# Autodesk Inventor assembly: Сборка
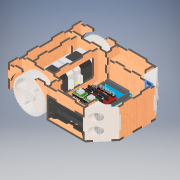
[picture p0: Inventor's stored thumbnail of the model, 180x180]
Saved by Autodesk Inventor 2019 (Build 230136000, 136)
## iProperties
Created: 2020-12-06
Part Number: Сборка
Material: Типовые
Document SubType Name: Assembly
Designer: Professional
Author: Professional
## Documents named in this file (25)
- C:\Users\Professional\Desktop\DeliveryBot\3dModels\assembly.iam
- C:\Users\Professional\Desktop\DeliveryBot\3dModels\Components\42BYGH47.ipt
- C:\Users\Professional\Desktop\DeliveryBot\3dModels\LaserCutter\base.ipt
- C:\Users\Professional\Desktop\DeliveryBot\3dModels\LaserCutter\top.ipt
- C:\Users\Professional\Desktop\DeliveryBot\3dModels\LaserCutter\batTop.ipt
- C:\Users\Professional\Desktop\DeliveryBot\3dModels\3DPrinter\Sensor_L.ipt
- C:\Users\Professional\Desktop\DeliveryBot\3dModels\LaserCutter\batMain.ipt
- C:\Users\Professional\Desktop\DeliveryBot\3dModels\LaserCutter\batBack.ipt
- C:\Users\Professional\Desktop\DeliveryBot\3dModels\LaserCutter\batN.ipt
- C:\Users\Professional\Desktop\DeliveryBot\3dModels\3DPrinter\Sensor_R.ipt
- C:\Users\Professional\Desktop\DeliveryBot\3dModels\LaserCutter\spacer.ipt
- C:\Users\Professional\Desktop\DeliveryBot\3dModels\LaserCutter\stepperMount.ipt
- C:\Users\Professional\Desktop\DeliveryBot\3dModels\LaserCutter\stiffenerFront.ipt
- C:\Users\Professional\Desktop\DeliveryBot\3dModels\LaserCutter\stiffenerBack.ipt
- C:\Users\Professional\Desktop\DeliveryBot\3dModels\3DPrinter\sameSpacer.ipt
- C:\Users\Professional\Desktop\DeliveryBot\3dModels\LaserCutter\back.ipt
- C:\Users\Professional\Desktop\DeliveryBot\3dModels\3DPrinter\wheel_L.ipt
- C:\Users\Professional\Desktop\DeliveryBot\3dModels\3DPrinter\wheel_R.ipt
- C:\Users\Professional\Desktop\DeliveryBot\3dModels\LaserCutter\protector.ipt
- C:\Users\Professional\Desktop\DeliveryBot\3dModels\components\HC-SR04.ipt
- C:\Users\Professional\Desktop\DeliveryBot\3dModels\Components\ArduinoMega.ipt
- C:\Users\Professional\Desktop\DeliveryBot\3dModels\components\CNC shield.ipt
- C:\Users\Professional\Desktop\DeliveryBot\3dModels\Components\2x18650 holder.ipt
- C:\Users\Professional\Desktop\DeliveryBot\3dModels\components\smallWheel.ipt
- C:\Users\Professional\Desktop\DeliveryBot\3dModels\3DPrinter\smallWheelStator.ipt
## Components (35 placed, 24 different names)
1. 42BYGH47:1 — Угол:1, Жесткий:24, С поворотом:2
2. base:1 — Жесткий:1, Жесткий:4, Жесткий:6, Жесткий:8, Жесткий:9, Жесткий:10, Жесткий:11, Жесткий:12, Жесткий:18, Жесткий:19, Жесткий:22, Жесткий:23, Жесткий:37, Жесткий:38
3. top:1 — Жесткий:1, Жесткий:14
4. 42BYGH47:2 — Угол:1, Жесткий:25, С поворотом:1
5. batTop:1 — Жесткий:8, Жесткий:13
6. batTop:2 — Жесткий:4, Жесткий:15
7. Sensor_L:2 — Жесткий:6, Жесткий:33
8. batMain:1 — Жесткий:10, Жесткий:35
9. batMain:2 — Жесткий:9, Жесткий:36
10. batBack:1 — Жесткий:11
11. batBack:2 — Жесткий:12
12. batN:1 — Жесткий:13, Жесткий:16
13. batN:2 — Жесткий:15, Жесткий:28
14. Sensor_R:1 — Жесткий:14, Жесткий:34
15. spacer:1 — Жесткий:16
16. stepperMount:1 — Жесткий:19, Жесткий:24
17. stepperMount:2 — Жесткий:18, Жесткий:25
18. stiffenerFront:1 — Жесткий:22
19. stiffenerBack:1 — Жесткий:23, Жесткий:31
20. back:1 — Жесткий:29, Жесткий:30, Жесткий:39
21. wheel_L:2 — С поворотом:1
22. wheel_R:1 — С поворотом:2
23. spacer:2 — Жесткий:28
24. protector:1 — Жесткий:29
25. protector:2 — Жесткий:30
26. sameSpacer:1 — Жесткий:31, Жесткий:39
27. HC-SR04:1 — Жесткий:33
28. HC-SR04:2 — Жесткий:34
29. ArduinoMega:1
30. CNC shield:1
31. 2x18650 holder:1 — Жесткий:35
32. 2x18650 holder:2 — Жесткий:36
33. smallWheel:1 — С поворотом:3
34. smallWheelStator:1 — Жесткий:38
35. smallWheelStator:2 — Жесткий:37, С поворотом:3
## Relationships (33: WeldJoint 29, RevoluteJoint 3, Angle 1)
- Жесткий:1 [WeldJoint]: base:1 ↔ top:1
- Угол:1 [Angle] (180 deg): 42BYGH47:1 ↔ 42BYGH47:2
- Жесткий:4 [WeldJoint]: base:1 ↔ batTop:2
- Жесткий:6 [WeldJoint]: base:1 ↔ Sensor_L:2
- Жесткий:8 [WeldJoint]: base:1 ↔ batTop:1
- Жесткий:9 [WeldJoint]: base:1 ↔ batMain:2
- Жесткий:10 [WeldJoint]: base:1 ↔ batMain:1
- Жесткий:11 [WeldJoint]: base:1 ↔ batBack:1
- Жесткий:12 [WeldJoint]: base:1 ↔ batBack:2
- Жесткий:13 [WeldJoint]: batTop:1 ↔ batN:1
- Жесткий:14 [WeldJoint]: top:1 ↔ Sensor_R:1
- Жесткий:15 [WeldJoint]: batTop:2 ↔ batN:2
- Жесткий:16 [WeldJoint]: batN:1 ↔ spacer:1
- Жесткий:18 [WeldJoint]: base:1 ↔ stepperMount:2
- Жесткий:19 [WeldJoint]: base:1 ↔ stepperMount:1
- Жесткий:22 [WeldJoint]: base:1 ↔ stiffenerFront:1
- Жесткий:23 [WeldJoint]: base:1 ↔ stiffenerBack:1
- Жесткий:24 [WeldJoint]: 42BYGH47:1 ↔ stepperMount:1
- Жесткий:25 [WeldJoint]: 42BYGH47:2 ↔ stepperMount:2
- С поворотом:1 [RevoluteJoint] (-19 mm): 42BYGH47:2 ↔ wheel_L:2
- С поворотом:2 [RevoluteJoint] (-19 mm): 42BYGH47:1 ↔ wheel_R:1
- Жесткий:28 [WeldJoint]: batN:2 ↔ spacer:2
- Жесткий:29 [WeldJoint]: back:1 ↔ protector:1
- Жесткий:30 [WeldJoint]: back:1 ↔ protector:2
- Жесткий:31 [WeldJoint]: stiffenerBack:1 ↔ sameSpacer:1
- Жесткий:33 [WeldJoint]: Sensor_L:2 ↔ HC-SR04:1
- Жесткий:34 [WeldJoint]: Sensor_R:1 ↔ HC-SR04:2
- Жесткий:35 [WeldJoint]: batMain:1 ↔ 2x18650 holder:1
- Жесткий:36 [WeldJoint]: batMain:2 ↔ 2x18650 holder:2
- Жесткий:37 [WeldJoint]: base:1 ↔ smallWheelStator:2
- Жесткий:38 [WeldJoint]: base:1 ↔ smallWheelStator:1
- С поворотом:3 [RevoluteJoint]: smallWheel:1 ↔ smallWheelStator:2
- Жесткий:39 [WeldJoint]: back:1 ↔ sameSpacer:1
